# Autodesk Inventor assembly: FullField-ver6-1111-2021
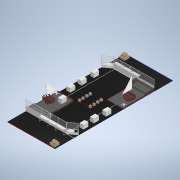
[picture p0: Inventor's stored thumbnail of the model, 180x180]
Saved by Autodesk Inventor 2021 (Build 250183000, 183)
## iProperties
Created: 2021-02-23
Part Number: FullField-ver6-1111-2021
Document SubType Name: Assembly
Designer: CMurray
Author: CMurray
## Documents named in this file (22)
- F:\PHRC CADD 2021\2021 Game Design Challenge\Full Field\Final Assembly\FullField-ver6-1111-2021.iam
- F:\PHRC CADD 2021\2021 Game Design Challenge\Full Field\Parts\FieldFloor-ver1-1111-2021.ipt
- F:\PHRC CADD 2021\2021 Game Design Challenge\Full Field\Parts\Tape\Tape.ipt
- F:\PHRC CADD 2021\2021 Game Design Challenge\Full Field\Parts\Tape\RedAllianceTape-ver1-1111-2021.ipt
- F:\PHRC CADD 2021\2021 Game Design Challenge\Full Field\Parts\Tape\BlueAllianceTape-ver1-1111-2021.ipt
- F:\PHRC CADD 2021\2021 Game Design Challenge\Player Station\Assemblies\DriverStation-ver2-1111-2021.iam
- F:\PHRC CADD 2021\2021 Game Design Challenge\Crow's Nest\Assemblies\CrowsNestFinal-ver3-1111-2021.iam
- F:\PHRC CADD 2021\2021 Game Design Challenge\Misc\MockRobot-ver1-1111-2021.ipt
- F:\PHRC CADD 2021\2021 Game Design Challenge\Main Ship\RedShip-ver1-1111-2021.ipt
- F:\PHRC CADD 2021\2021 Game Design Challenge\Crow's Nest\Parts\Capstan\test.ipt
- F:\PHRC CADD 2021\2021 Game Design Challenge\Crow's Nest\Parts\Capstan\CapTop-ver1-1111-2021.ipt
- F:\PHRC CADD 2021\2021 Game Design Challenge\Crow's Nest\Parts\Capstan\FullSailCapstan-ver2-1111-2021.iam
- F:\PHRC CADD 2021\2021 Game Design Challenge\Full Field\Parts\Tape\Tape2.ipt
- F:\PHRC CADD 2021\2021 Game Design Challenge\Main Ship\BlueShip-ver1-1111-2021.ipt
- F:\PHRC CADD 2021\2021 Game Design Challenge\Crow's Nest\Assemblies\BlueCrowsNestFinal-ver1-1111-2021.iam
- F:\PHRC CADD 2021\2021 Game Design Challenge\Misc\cargoPrototype.ipt
- F:\PHRC CADD 2021\2021 Game Design Challenge\Full Field\Parts\Tape\MidSquareFull.iam
- F:\PHRC CADD 2021\2021 Game Design Challenge\Treasure Chest\PTreasureChestFinal-ver1-1111-2021.ipt
- F:\PHRC CADD 2021\2021 Game Design Challenge\Full Field\Parts\Tape\RedAllianceTape-ver2-1111-2021.ipt
- F:\PHRC CADD 2021\2021 Game Design Challenge\Full Field\Parts\Tape\BlueAllianceTape-ver2-1111-2021.ipt
- F:\PHRC CADD 2021\2021 Game Design Challenge\Anchor\CapstanBottom-ver1-1111-2021.ipt
- F:\PHRC CADD 2021\2021 Game Design Challenge\Anchor\CapstanTop-ver1-1111-2021.ipt
## Components (72 placed, 21 different names)
1. FieldFloor-ver1-1111-2021:1 — Flush:1, Flush:2, Mate:1, Mate:3, Mate:10, Flush:10, Mate:14, Flush:12, Mate:32, Mate:34, Mate:51, Flush:24, Mate:53, Flush:25, Mate:63, Mate:69, Mate:70, Mate:71, Mate:75, Mate:76, Mate:88, Flush:26, Mate:104, Mate:105, Mate:106, Mate:107, Mate:108, Mate:109, Mate:110, Mate:111, Mate:112, Flush:30
2. FieldFloor-ver1-1111-2021:2 — Flush:1, Flush:2, Mate:1, Mate:2, Flush:3, Flush:4, Flush:5, Flush:6, Mate:8, Flush:9, Mate:12, Flush:11, Flush:19, Mate:36, Flush:20, Mate:49, Flush:23, Mate:62, Mate:66, Mate:67, Mate:68, Mate:72, Mate:77, Mate:78, Mate:79, Mate:80, Mate:83, Mate:85, Flush:27, Mate:89, Flush:28, Flush:29, Mate:90, Mate:91, Mate:92, Mate:93, Mate:94, Mate:95, Mate:96, Mate:97, Mate:98
3. BlueAllianceTape-ver2-1111-2021:1 — Mate:89, Flush:28, Flush:29
4. RedAllianceTape-ver2-1111-2021:1 — Mate:88, Flush:26, Flush:27
5. MidSquareFull:1 [sub-assembly] — Mate:72, Mate:73, Mate:74
6. Tape2:1 — Mate:49, Flush:23, Mate:50
7. Tape2:2 — Mate:51, Flush:24, Mate:52, Mate:73
8. Tape:1 — Mate:2, Flush:3, Flush:4, Mate:9, Mate:11, Mate:33, Mate:50, Mate:74, Mate:87
9. Tape:2 — Mate:3, Flush:5, Flush:6, Mate:13, Mate:15, Mate:35, Mate:52, Mate:84
10. RedAllianceTape-ver1-1111-2021:1 — Mate:8, Flush:9, Mate:9
11. RedAllianceTape-ver1-1111-2021:2 — Mate:10, Flush:10, Mate:11
12. BlueAllianceTape-ver1-1111-2021:1 — Mate:12, Flush:11, Mate:13
13. BlueAllianceTape-ver1-1111-2021:2 — Mate:14, Flush:12, Mate:15
14. CapstanBottom-ver1-1111-2021:1 — Mate:117, Rotational:5, Flush:31, Flush:32
15. CapstanTop-ver1-1111-2021:1 — Rotational:5
16. CapTop-ver1-1111-2021:2
17. FullSailCapstan-ver2-1111-2021:3 [sub-assembly] — Rotational:4
18. test:2 — Mate:57, Mate:58, Mate:59, Rotational:4
19. BlueShip-ver1-1111-2021:1 — Mate:53, Mate:54, Flush:25, Mate:55, Mate:56, Mate:86, Mate:117, Flush:31, Flush:32
20. BlueCrowsNestFinal-ver1-1111-2021:1 [sub-assembly] — Mate:55, Mate:56, Mate:57, Mate:58, Mate:59
21. CapstanBottom-ver1-1111-2021:2 — Mate:118, Mate:119, Mate:120
22. CapstanTop-ver1-1111-2021:2
23. CapTop-ver1-1111-2021:1 — Rotational:2
24. FullSailCapstan-ver2-1111-2021:2 [sub-assembly] — Rotational:1, Rotational:2
25. test:1 — Mate:41, Flush:21, Mate:42, Rotational:1
26. RedShip-ver1-1111-2021:1 — Mate:36, Mate:37, Flush:20, Mate:38, Mate:40, Mate:81, Mate:82, Mate:118, Mate:119, Mate:120
27. CrowsNestFinal-ver3-1111-2021:1 [sub-assembly] — Mate:38, Mate:40, Mate:41, Flush:21, Mate:42
28. DriverStation-ver2-1111-2021:2 [sub-assembly] — Mate:34, Mate:35, Flush:19, Mate:37
29. DriverStation-ver2-1111-2021:1 [sub-assembly] — Mate:32, Mate:33, Mate:54, Flush:30
30. cargoPrototype:9 — Mate:90
31. cargoPrototype:10 — Mate:91
32. cargoPrototype:11 — Mate:92
33. cargoPrototype:12 — Mate:93, Mate:99, Mate:100, Mate:102
34. cargoPrototype:13 — Mate:94, Mate:103
35. cargoPrototype:14 — Mate:95
36. cargoPrototype:15 — Mate:96
37. cargoPrototype:16 — Mate:97, Mate:101
38. cargoPrototype:17 — Mate:98
39. cargoPrototype:18 — Mate:99, Mate:100
40. cargoPrototype:19 — Mate:101
41. cargoPrototype:20 — Mate:102
42. cargoPrototype:21 — Mate:103
43. cargoPrototype:22 — Mate:110
44. cargoPrototype:23 — Mate:112, Mate:113
45. cargoPrototype:24 — Mate:108, Mate:114
46. cargoPrototype:25 — Mate:111
47. cargoPrototype:26 — Mate:107
48. cargoPrototype:27 — Mate:106
49. cargoPrototype:28 — Mate:109
50. cargoPrototype:29 — Mate:105
51. cargoPrototype:30 — Mate:104, Mate:115, Mate:116
52. cargoPrototype:31 — Mate:113
53. cargoPrototype:32 — Mate:114
54. cargoPrototype:33 — Mate:115
55. cargoPrototype:34 — Mate:116
56. cargoPrototype:2 — Mate:63
57. cargoPrototype:3 — Mate:75
58. cargoPrototype:4 — Mate:76
59. cargoPrototype:5 — Mate:78
60. cargoPrototype:6 — Mate:77
61. cargoPrototype:7 — Mate:79
62. cargoPrototype:8 — Mate:80
63. cargoPrototype:1 — Mate:62
64. PTreasureChestFinal-ver1-1111-2021:1 — Mate:82, Mate:83, Mate:84
65. PTreasureChestFinal-ver1-1111-2021:2 — Mate:85, Mate:86, Mate:87
66. MockRobot-ver1-1111-2021:8 — Mate:81
67. MockRobot-ver1-1111-2021:1 — Mate:66
68. MockRobot-ver1-1111-2021:3 — Mate:67
69. MockRobot-ver1-1111-2021:4 — Mate:68
70. MockRobot-ver1-1111-2021:5 — Mate:69
71. MockRobot-ver1-1111-2021:6 — Mate:70
72. MockRobot-ver1-1111-2021:7 — Mate:71
## Relationships (118: Mate 89, Flush 23, RevoluteJoint 6)
- Flush:1: FieldFloor-ver1-1111-2021:1 ↔ FieldFloor-ver1-1111-2021:2
- Flush:2: FieldFloor-ver1-1111-2021:1 ↔ FieldFloor-ver1-1111-2021:2
- Mate:1: FieldFloor-ver1-1111-2021:1 ↔ FieldFloor-ver1-1111-2021:2
- Mate:2: FieldFloor-ver1-1111-2021:2 ↔ Tape:1
- Flush:3: FieldFloor-ver1-1111-2021:2 ↔ Tape:1
- Flush:4 (3606.8 mm): FieldFloor-ver1-1111-2021:2 ↔ Tape:1
- Mate:3: FieldFloor-ver1-1111-2021:1 ↔ Tape:2
- Flush:5: FieldFloor-ver1-1111-2021:2 ↔ Tape:2
- Flush:6 (3606.8 mm): FieldFloor-ver1-1111-2021:2 ↔ Tape:2
- Mate:8: FieldFloor-ver1-1111-2021:2 ↔ RedAllianceTape-ver1-1111-2021:1
- Flush:9: FieldFloor-ver1-1111-2021:2 ↔ RedAllianceTape-ver1-1111-2021:1
- Mate:9: Tape:1 ↔ RedAllianceTape-ver1-1111-2021:1
- Mate:10: FieldFloor-ver1-1111-2021:1 ↔ RedAllianceTape-ver1-1111-2021:2
- Flush:10: FieldFloor-ver1-1111-2021:1 ↔ RedAllianceTape-ver1-1111-2021:2
- Mate:11: Tape:1 ↔ RedAllianceTape-ver1-1111-2021:2
- Mate:12: FieldFloor-ver1-1111-2021:2 ↔ BlueAllianceTape-ver1-1111-2021:1
- Flush:11: FieldFloor-ver1-1111-2021:2 ↔ BlueAllianceTape-ver1-1111-2021:1
- Mate:13: Tape:2 ↔ BlueAllianceTape-ver1-1111-2021:1
- Mate:14: FieldFloor-ver1-1111-2021:1 ↔ BlueAllianceTape-ver1-1111-2021:2
- Flush:12: FieldFloor-ver1-1111-2021:1 ↔ BlueAllianceTape-ver1-1111-2021:2
- Mate:15: Tape:2 ↔ BlueAllianceTape-ver1-1111-2021:2
- Mate:32: FieldFloor-ver1-1111-2021:1 ↔ DriverStation-ver2-1111-2021:1
- Mate:33: Tape:1 ↔ DriverStation-ver2-1111-2021:1
- Mate:34: FieldFloor-ver1-1111-2021:1 ↔ DriverStation-ver2-1111-2021:2
- Mate:35: Tape:2 ↔ DriverStation-ver2-1111-2021:2
- Flush:19: FieldFloor-ver1-1111-2021:2 ↔ DriverStation-ver2-1111-2021:2
- Mate:36: FieldFloor-ver1-1111-2021:2 ↔ RedShip-ver1-1111-2021:1
- Mate:37: RedShip-ver1-1111-2021:1 ↔ DriverStation-ver2-1111-2021:2
- Flush:20: FieldFloor-ver1-1111-2021:2 ↔ RedShip-ver1-1111-2021:1
- Mate:38: RedShip-ver1-1111-2021:1 ↔ CrowsNestFinal-ver3-1111-2021:1
- Mate:40 (1778 mm): RedShip-ver1-1111-2021:1 ↔ CrowsNestFinal-ver3-1111-2021:1
- Mate:41: test:1 ↔ CrowsNestFinal-ver3-1111-2021:1
- Flush:21 (-203.2 mm): test:1 ↔ CrowsNestFinal-ver3-1111-2021:1
- Mate:42 (762 mm): test:1 ↔ CrowsNestFinal-ver3-1111-2021:1
- Rotational:1 [RevoluteJoint]: FullSailCapstan-ver2-1111-2021:2 ↔ test:1
- Rotational:2 [RevoluteJoint]: CapTop-ver1-1111-2021:1 ↔ FullSailCapstan-ver2-1111-2021:2
- Mate:49: FieldFloor-ver1-1111-2021:2 ↔ Tape2:1
- Flush:23 (1524 mm): FieldFloor-ver1-1111-2021:2 ↔ Tape2:1
- Mate:50: Tape2:1 ↔ Tape:1
- Mate:51: FieldFloor-ver1-1111-2021:1 ↔ Tape2:2
- Flush:24 (1524 mm): FieldFloor-ver1-1111-2021:1 ↔ Tape2:2
- Mate:52: Tape2:2 ↔ Tape:2
- Mate:53: FieldFloor-ver1-1111-2021:1 ↔ BlueShip-ver1-1111-2021:1
- Mate:54: BlueShip-ver1-1111-2021:1 ↔ DriverStation-ver2-1111-2021:1
- Flush:25: FieldFloor-ver1-1111-2021:1 ↔ BlueShip-ver1-1111-2021:1
- Mate:55: BlueShip-ver1-1111-2021:1 ↔ BlueCrowsNestFinal-ver1-1111-2021:1
- Mate:56 (1397 mm): BlueShip-ver1-1111-2021:1 ↔ BlueCrowsNestFinal-ver1-1111-2021:1
- Mate:57: test:2 ↔ BlueCrowsNestFinal-ver1-1111-2021:1
- Mate:58 (-203.2 mm): test:2 ↔ BlueCrowsNestFinal-ver1-1111-2021:1
- Mate:59 (762 mm): test:2 ↔ BlueCrowsNestFinal-ver1-1111-2021:1
- [RevoluteJoint]: CapTop-ver1-1111-2021:2 ↔ FullSailCapstan-ver2-1111-2021:3
- Rotational:4 [RevoluteJoint]: FullSailCapstan-ver2-1111-2021:3 ↔ test:2
- Mate:62: FieldFloor-ver1-1111-2021:2 ↔ cargoPrototype:1
- Mate:63: FieldFloor-ver1-1111-2021:1 ↔ cargoPrototype:2
- Mate:66: FieldFloor-ver1-1111-2021:2 ↔ MockRobot-ver1-1111-2021:1
- Mate:67: FieldFloor-ver1-1111-2021:2 ↔ MockRobot-ver1-1111-2021:3
- Mate:68: FieldFloor-ver1-1111-2021:2 ↔ MockRobot-ver1-1111-2021:4
- Mate:69: FieldFloor-ver1-1111-2021:1 ↔ MockRobot-ver1-1111-2021:5
- Mate:70: FieldFloor-ver1-1111-2021:1 ↔ MockRobot-ver1-1111-2021:6
- Mate:71: FieldFloor-ver1-1111-2021:1 ↔ MockRobot-ver1-1111-2021:7
- Mate:72: FieldFloor-ver1-1111-2021:2 ↔ MidSquareFull:1
- Mate:73 (1930.4 mm): MidSquareFull:1 ↔ Tape2:2
- Mate:74 (6553.2 mm): MidSquareFull:1 ↔ Tape:1
- Mate:75: FieldFloor-ver1-1111-2021:1 ↔ cargoPrototype:3
- Mate:76: FieldFloor-ver1-1111-2021:1 ↔ cargoPrototype:4
- Mate:77: FieldFloor-ver1-1111-2021:2 ↔ cargoPrototype:6
- Mate:78: FieldFloor-ver1-1111-2021:2 ↔ cargoPrototype:5
- Mate:79: FieldFloor-ver1-1111-2021:2 ↔ cargoPrototype:7
- Mate:80: FieldFloor-ver1-1111-2021:2 ↔ cargoPrototype:8
- Mate:81: RedShip-ver1-1111-2021:1 ↔ MockRobot-ver1-1111-2021:8
- Mate:82 (25.4 mm): RedShip-ver1-1111-2021:1 ↔ PTreasureChestFinal-ver1-1111-2021:1
- Mate:83: FieldFloor-ver1-1111-2021:2 ↔ PTreasureChestFinal-ver1-1111-2021:1
- Mate:84: Tape:2 ↔ PTreasureChestFinal-ver1-1111-2021:1
- Mate:85: FieldFloor-ver1-1111-2021:2 ↔ PTreasureChestFinal-ver1-1111-2021:2
- Mate:86 (25.4 mm): BlueShip-ver1-1111-2021:1 ↔ PTreasureChestFinal-ver1-1111-2021:2
- Mate:87: Tape:1 ↔ PTreasureChestFinal-ver1-1111-2021:2
- Mate:88: FieldFloor-ver1-1111-2021:1 ↔ RedAllianceTape-ver2-1111-2021:1
- Flush:26: FieldFloor-ver1-1111-2021:1 ↔ RedAllianceTape-ver2-1111-2021:1
- Flush:27: FieldFloor-ver1-1111-2021:2 ↔ RedAllianceTape-ver2-1111-2021:1
- Mate:89: FieldFloor-ver1-1111-2021:2 ↔ BlueAllianceTape-ver2-1111-2021:1
- Flush:28: FieldFloor-ver1-1111-2021:2 ↔ BlueAllianceTape-ver2-1111-2021:1
- Flush:29: FieldFloor-ver1-1111-2021:2 ↔ BlueAllianceTape-ver2-1111-2021:1
- Mate:90: FieldFloor-ver1-1111-2021:2 ↔ cargoPrototype:9
- Mate:91: FieldFloor-ver1-1111-2021:2 ↔ cargoPrototype:10
- Mate:92: FieldFloor-ver1-1111-2021:2 ↔ cargoPrototype:11
- Mate:93: FieldFloor-ver1-1111-2021:2 ↔ cargoPrototype:12
- Mate:94: FieldFloor-ver1-1111-2021:2 ↔ cargoPrototype:13
- Mate:95: FieldFloor-ver1-1111-2021:2 ↔ cargoPrototype:14
- Mate:96: FieldFloor-ver1-1111-2021:2 ↔ cargoPrototype:15
- Mate:97: FieldFloor-ver1-1111-2021:2 ↔ cargoPrototype:16
- Mate:98: FieldFloor-ver1-1111-2021:2 ↔ cargoPrototype:17
- Mate:99: cargoPrototype:12 ↔ cargoPrototype:18
- Mate:100: cargoPrototype:12 ↔ cargoPrototype:18
- Mate:101: cargoPrototype:16 ↔ cargoPrototype:19
- Mate:102: cargoPrototype:12 ↔ cargoPrototype:20
- Mate:103: cargoPrototype:13 ↔ cargoPrototype:21
- Mate:104: FieldFloor-ver1-1111-2021:1 ↔ cargoPrototype:30
- Mate:105: FieldFloor-ver1-1111-2021:1 ↔ cargoPrototype:29
- Mate:106: FieldFloor-ver1-1111-2021:1 ↔ cargoPrototype:27
- Mate:107: FieldFloor-ver1-1111-2021:1 ↔ cargoPrototype:26
- Mate:108: FieldFloor-ver1-1111-2021:1 ↔ cargoPrototype:24
- Mate:109: FieldFloor-ver1-1111-2021:1 ↔ cargoPrototype:28
- Mate:110: FieldFloor-ver1-1111-2021:1 ↔ cargoPrototype:22
- Mate:111: FieldFloor-ver1-1111-2021:1 ↔ cargoPrototype:25
- Mate:112: FieldFloor-ver1-1111-2021:1 ↔ cargoPrototype:23
- Mate:113: cargoPrototype:23 ↔ cargoPrototype:31
- Mate:114: cargoPrototype:24 ↔ cargoPrototype:32
- Mate:115: cargoPrototype:30 ↔ cargoPrototype:33
- Mate:116: cargoPrototype:30 ↔ cargoPrototype:34
- Flush:30: FieldFloor-ver1-1111-2021:1 ↔ DriverStation-ver2-1111-2021:1
- Mate:117: CapstanBottom-ver1-1111-2021:1 ↔ BlueShip-ver1-1111-2021:1
- Rotational:5 [RevoluteJoint]: CapstanBottom-ver1-1111-2021:1 ↔ CapstanTop-ver1-1111-2021:1
- Flush:31 (-3937 mm): CapstanBottom-ver1-1111-2021:1 ↔ BlueShip-ver1-1111-2021:1
- Flush:32 (-304.8 mm): CapstanBottom-ver1-1111-2021:1 ↔ BlueShip-ver1-1111-2021:1
- [RevoluteJoint]: CapstanBottom-ver1-1111-2021:2 ↔ CapstanTop-ver1-1111-2021:2
- Mate:118: CapstanBottom-ver1-1111-2021:2 ↔ RedShip-ver1-1111-2021:1
- Mate:119 (3937 mm): CapstanBottom-ver1-1111-2021:2 ↔ RedShip-ver1-1111-2021:1
- Mate:120 (304.8 mm): CapstanBottom-ver1-1111-2021:2 ↔ RedShip-ver1-1111-2021:1
## Named parameters: d150_d121 = 0 mm, d151_d122 = 10.074303 deg, d236_d232 = 0 mm, d237_d233 = 135.645569 deg
